# Autodesk Inventor assembly: BuczekSumowksi
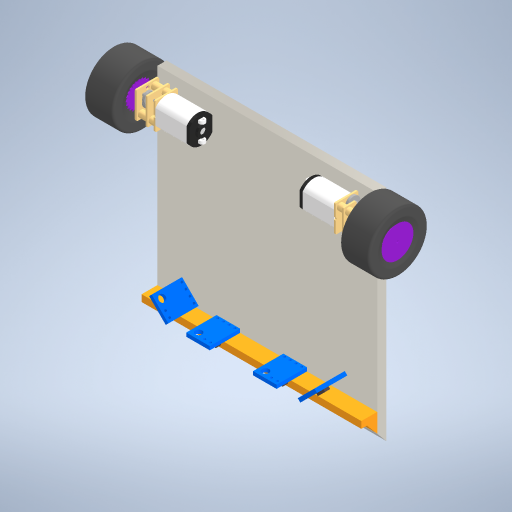
[picture p0: Inventor's stored thumbnail of the model, 512x512]
Saved by Autodesk Inventor 2023 (Build 270158000, 158)
## iProperties
Created: 2024-03-04
Part Number: BuczekSumowksi
Document SubType Name: Assembly
Designer: pavel
Author: pavel
## Documents named in this file (7)
- C:\Users\pavel\Documents\BuczekSumowski\BuczekSumowskiMechanics\BuczekSumowksi.iam
- C:\Users\pavel\Documents\BuczekSumowski\BuczekSumowskiMechanics\MetalBottom.ipt
- C:\Users\pavel\Documents\BuczekSumowski\BuczekSumowskiMechanics\vl53l0x.ipt
- C:\Users\pavel\Documents\BuczekSumowski\BuczekSumowskiMechanics\PlasticBody.ipt
- C:\Users\pavel\Documents\BuczekSumowski\BuczekSumowskiMechanics\MicroGearMotor Spool v2.iam
- C:\Users\pavel\Documents\BuczekSumowski\BuczekSumowskiMechanics\Wheel.ipt
- C:\Users\pavel\Documents\BuczekSumowski\BuczekSumowskiMechanics\Buczek Sumowski - kolo v2.ipt
## Components (12 placed, 6 different names)
1. MetalBottom:1 — Mate:1, Angle:1, Mate:3, Mate:4, Angle:2, Mate:5, Mate:8, Mate:9, Flush:1, Flush:2, Flush:3, Mate:14, Mate:15
2. vl53l0x:2 — Mate:3, Mate:7, Mate:10
3. vl53l0x:5 — Mate:5, Mate:6, Mate:10, Flush:3
4. vl53l0x:3 — Mate:1, Angle:1, Mate:12, Mate:14
5. vl53l0x:4 — Mate:4, Angle:2, Mate:13, Mate:15
6. PlasticBody:1 — Mate:6, Mate:7, Mate:12, Mate:13
7. MicroGearMotor Spool v2:1 [sub-assembly] — Mate:8, Flush:2, Mate:21, Mate:22, Mate:23, Mate:25
8. MicroGearMotor Spool v2:2 [sub-assembly] — Mate:9, Flush:1, Mate:16, Mate:17, Mate:18, Mate:20
9. Wheel:1 — Mate:23, Mate:24, Mate:25
10. Wheel:2 — Mate:18, Mate:19, Mate:20
11. Buczek Sumowski - kolo v2:1 — Mate:16, Mate:17, Mate:19
12. Buczek Sumowski - kolo v2:2 — Mate:21, Mate:22, Mate:24
## Relationships (28: Mate 23, Flush 3, Angle 2)
- Mate:1: MetalBottom:1 ↔ vl53l0x:3
- Angle:1 (-45 deg): MetalBottom:1 ↔ vl53l0x:3
- Mate:3: MetalBottom:1 ↔ vl53l0x:2
- Mate:4: MetalBottom:1 ↔ vl53l0x:4
- Angle:2 (-45 deg): MetalBottom:1 ↔ vl53l0x:4
- Mate:5: MetalBottom:1 ↔ vl53l0x:5
- Mate:6: vl53l0x:5 ↔ PlasticBody:1
- Mate:7: vl53l0x:2 ↔ PlasticBody:1
- Mate:8: MetalBottom:1 ↔ MicroGearMotor Spool v2:1
- Mate:9: MetalBottom:1 ↔ MicroGearMotor Spool v2:2
- Flush:1: MetalBottom:1 ↔ MicroGearMotor Spool v2:2
- Flush:2: MetalBottom:1 ↔ MicroGearMotor Spool v2:1
- Mate:10 (25 mm): vl53l0x:2 ↔ vl53l0x:5
- Mate:12: vl53l0x:3 ↔ PlasticBody:1
- Mate:13: vl53l0x:4 ↔ PlasticBody:1
- Flush:3 (31.5 mm): MetalBottom:1 ↔ vl53l0x:5
- Mate:14 (-16 mm): MetalBottom:1 ↔ vl53l0x:3
- Mate:15 (-16 mm): MetalBottom:1 ↔ vl53l0x:4
- Mate:16: MicroGearMotor Spool v2:2 ↔ Buczek Sumowski - kolo v2:1
- Mate:17: MicroGearMotor Spool v2:2 ↔ Buczek Sumowski - kolo v2:1
- Mate:18: MicroGearMotor Spool v2:2 ↔ Wheel:2
- Mate:19 (0.5 mm): Wheel:2 ↔ Buczek Sumowski - kolo v2:1
- Mate:20 (1.5 mm): MicroGearMotor Spool v2:2 ↔ Wheel:2
- Mate:21: MicroGearMotor Spool v2:1 ↔ Buczek Sumowski - kolo v2:2
- Mate:22: MicroGearMotor Spool v2:1 ↔ Buczek Sumowski - kolo v2:2
- Mate:23: MicroGearMotor Spool v2:1 ↔ Wheel:1
- Mate:24 (0.5 mm): Wheel:1 ↔ Buczek Sumowski - kolo v2:2
- Mate:25 (1.5 mm): MicroGearMotor Spool v2:1 ↔ Wheel:1
